# Autodesk Inventor assembly: Line Sensor
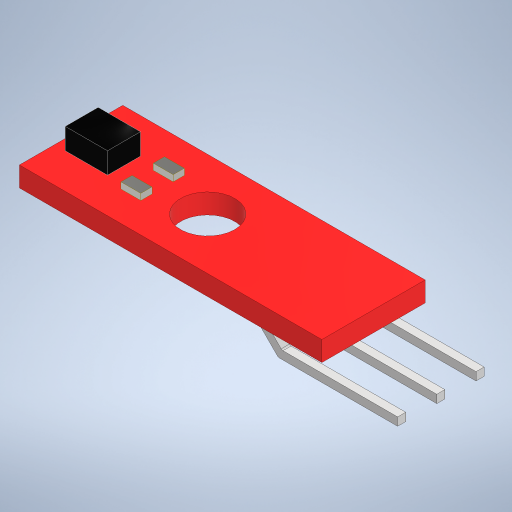
[picture p0: Inventor's stored thumbnail of the model, 512x512]
Saved by Autodesk Inventor 2023 (Build 270158000, 158)
## iProperties
Created: 2023-01-17
Part Number: Line Sensor
Document SubType Name: Assembly
Designer: remoh
Author: remoh
## Documents named in this file (5)
- C:\Users\remoh\Documents\HF Maschinenbau\AüP\Roboter CAD\Roboter CAD\V6\Infrarotsensor\Line Sensor.iam
- C:\Users\remoh\Documents\HF Maschinenbau\AüP\Roboter CAD\Roboter CAD\V6\Infrarotsensor\Grundplatte.ipt
- C:\Users\remoh\Documents\HF Maschinenbau\AüP\Roboter CAD\Roboter CAD\V6\Infrarotsensor\Sensor.ipt
- C:\Users\remoh\Documents\HF Maschinenbau\AüP\Roboter CAD\Roboter CAD\V6\Infrarotsensor\Widerstand 0603.ipt
- C:\Users\remoh\Documents\HF Maschinenbau\AüP\Roboter CAD\Roboter CAD\V6\Infrarotsensor\Pin.ipt
## Components (7 placed, 4 different names)
1. Grundplatte:1 — Passend:1, Fluchtend:1, Fluchtend:2, Passend:2, Passend:3, Fluchtend:3, Fluchtend:4, Fluchtend:5, Fluchtend:6, Passend:4, Passend:5, Fluchtend:7, Fluchtend:8, Passend:7, Passend:8
2. Sensor:1 — Passend:1, Fluchtend:1, Fluchtend:2
3. Widerstand 0603:1 — Passend:3, Fluchtend:4, Fluchtend:5
4. Widerstand 0603:2 — Passend:2, Fluchtend:3, Fluchtend:6
5. Pin:1 — Passend:4, Passend:5, Fluchtend:7, Passend:6, Fluchtend:9, Fluchtend:10
6. Pin:2 — Passend:6, Passend:7, Fluchtend:9
7. Pin:3 — Fluchtend:8, Passend:8, Fluchtend:10
## Relationships (18: Flush 10, Mate 8)
- Passend:1 [Mate]: Grundplatte:1 ↔ Sensor:1
- Fluchtend:1 [Flush] (0.85 mm): Grundplatte:1 ↔ Sensor:1
- Fluchtend:2 [Flush] (2.825 mm): Grundplatte:1 ↔ Sensor:1
- Passend:2 [Mate]: Grundplatte:1 ↔ Widerstand 0603:2
- Passend:3 [Mate]: Grundplatte:1 ↔ Widerstand 0603:1
- Fluchtend:3 [Flush] (2.4 mm): Grundplatte:1 ↔ Widerstand 0603:2
- Fluchtend:4 [Flush] (2.4 mm): Grundplatte:1 ↔ Widerstand 0603:1
- Fluchtend:5 [Flush] (5.75 mm): Grundplatte:1 ↔ Widerstand 0603:1
- Fluchtend:6 [Flush] (5.75 mm): Grundplatte:1 ↔ Widerstand 0603:2
- Passend:4 [Mate] (-7.3 mm): Grundplatte:1 ↔ Pin:1
- Passend:5 [Mate]: Grundplatte:1 ↔ Pin:1
- Fluchtend:7 [Flush] (-0.675 mm): Grundplatte:1 ↔ Pin:1
- Passend:6 [Mate] (2.5 mm): Pin:1 ↔ Pin:2
- Fluchtend:8 [Flush] (0.675 mm): Grundplatte:1 ↔ Pin:3
- Passend:7 [Mate]: Grundplatte:1 ↔ Pin:2
- Passend:8 [Mate]: Grundplatte:1 ↔ Pin:3
- Fluchtend:9 [Flush]: Pin:1 ↔ Pin:2
- Fluchtend:10 [Flush]: Pin:1 ↔ Pin:3
